# Autodesk Inventor assembly: Ensemble_Boite_chassis
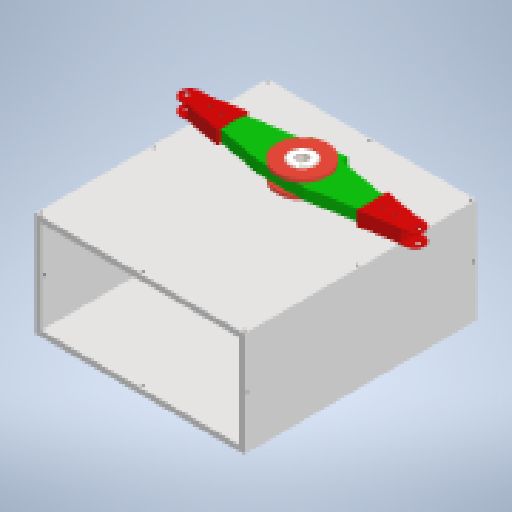
[picture p0: Inventor's stored thumbnail of the model, 512x512]
Saved by Autodesk Inventor 2025.2 (Build 292293000, 293)
## iProperties
Created: 2026-03-16
Part Number: Ensemble_Boite_chassis
Document SubType Name: Assembly
Designer: genon
Author: genon
## Documents named in this file (5)
- C:\Users\genon\Documents\Henallux Passerelle\Projet de conception\Cassini T-X\Inventor\Ensemble_Boite_chassis.iam
- C:\Users\genon\Documents\Henallux Passerelle\Projet de conception\Cassini T-X\Inventor\chassis_bas.ipt
- C:\Users\genon\Documents\Henallux Passerelle\Projet de conception\Cassini T-X\Inventor\chassis_côté.ipt
- C:\Users\genon\Documents\Henallux Passerelle\Projet de conception\Cassini T-X\Inventor\chassis_face_arriere.ipt
- C:\Users\genon\Documents\Henallux Passerelle\Projet de conception\Cassini T-X\Inventor\chassis_haut.ipt
## Components (6 placed, 4 different names)
1. chassis_bas:1 — Placage:1, Placage:2, Placage:3, Placage:4, Placage:5, Placage:7
2. chassis_côté:1 — Placage:1, Placage:2, Placage:6, Placage:8
3. chassis_côté:2 — Placage:3, Placage:4, Placage:9
4. chassis_face_arriere:1 — Placage:7, Placage:8
5. chassis_face_arriere:2 — Placage:5, Placage:6, Placage:10
6. chassis_haut:1 — Placage:9, Placage:10
## Relationships (10: Mate 10)
- Placage:1 [Mate]: chassis_bas:1 ↔ chassis_côté:1
- Placage:2 [Mate]: chassis_bas:1 ↔ chassis_côté:1
- Placage:3 [Mate]: chassis_bas:1 ↔ chassis_côté:2
- Placage:4 [Mate]: chassis_bas:1 ↔ chassis_côté:2
- Placage:5 [Mate]: chassis_bas:1 ↔ chassis_face_arriere:2
- Placage:6 [Mate]: chassis_côté:1 ↔ chassis_face_arriere:2
- Placage:7 [Mate]: chassis_bas:1 ↔ chassis_face_arriere:1
- Placage:8 [Mate]: chassis_côté:1 ↔ chassis_face_arriere:1
- Placage:9 [Mate]: chassis_côté:2 ↔ chassis_haut:1
- Placage:10 [Mate]: chassis_face_arriere:2 ↔ chassis_haut:1
